# Autodesk Inventor assembly: module_valve
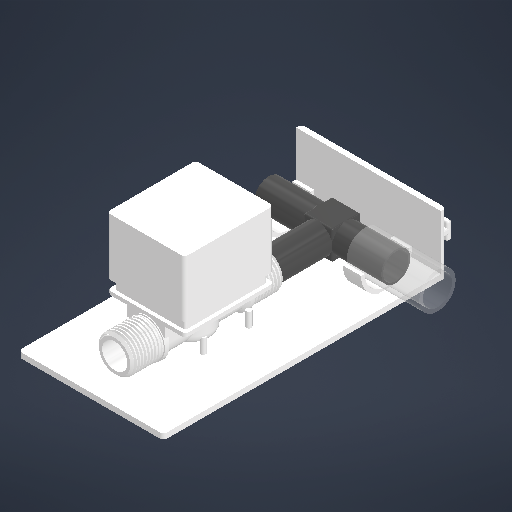
[picture p0: Inventor's stored thumbnail of the model, 512x512]
Saved by Autodesk Inventor 2025.4 (Build 294407000, 407)
## iProperties
Created: 2026-01-03
Part Number: module_valve
Document SubType Name: Assembly
Designer: sam
Author: sam
## Documents named in this file (6)
- G:\projects\primary\regulated-irrigation-system\model\asm\module-valve\module_valve.iam
- G:\projects\primary\regulated-irrigation-system\model\asm\electronic-components\valve-solenoid\valve-solenoid.iam
- G:\projects\primary\regulated-irrigation-system\model\asm\module-valve\module_valve.ipt
- G:\projects\primary\regulated-irrigation-system\model\asm\module-valve\t-piece_16.ipt
- G:\projects\primary\regulated-irrigation-system\model\asm\module-valve\clip-pipe.ipt
- G:\projects\primary\regulated-irrigation-system\model\asm\module-valve\pipe-16_flex-clear_stretched-over_40.ipt
## Components (6 placed, 5 different names)
1. valve-solenoid:1 [sub-assembly] — Mate:2, Mate:3, Angle:1
2. module_valve:1 — Mate:4, Mate:5, Mate:6, Mate:7, Mate:8, Mate:9, Flush:1, Angle:1, Flush:2
3. t-piece_16:1 — Mate:2, Mate:3, Mate:10, Flush:1, Mate:18
4. clip-pipe:1 — Mate:7, Mate:8, Mate:9
5. clip-pipe:2 — Mate:4, Mate:5, Mate:6, Mate:10
6. pipe-16_flex-clear_stretched-over_40:1 — Mate:18, Flush:2
## Relationships (13: Mate 10, Flush 2, Angle 1)
- Mate:2: valve-solenoid:1 ↔ t-piece_16:1
- Mate:3: valve-solenoid:1 ↔ t-piece_16:1
- Mate:4: module_valve:1 ↔ clip-pipe:2
- Mate:5: module_valve:1 ↔ clip-pipe:2
- Mate:6: module_valve:1 ↔ clip-pipe:2
- Mate:7: module_valve:1 ↔ clip-pipe:1
- Mate:8: module_valve:1 ↔ clip-pipe:1
- Mate:9: module_valve:1 ↔ clip-pipe:1
- Mate:10: t-piece_16:1 ↔ clip-pipe:2
- Flush:1 (3 mm): module_valve:1 ↔ t-piece_16:1
- Angle:1 (90 deg): valve-solenoid:1 ↔ module_valve:1
- Mate:18: t-piece_16:1 ↔ pipe-16_flex-clear_stretched-over_40:1
- Flush:2 (-20 mm): module_valve:1 ↔ pipe-16_flex-clear_stretched-over_40:1
